# Autodesk Inventor assembly: Geeetech GT9S2 Extruder
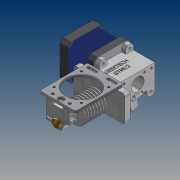
[picture p0: Inventor's stored thumbnail of the model, 180x180]
Saved by Autodesk Inventor 2019 (Build 230136000, 136)
## iProperties
Created: 2018-11-15
Part Number: Geeetech GT9S2 Extruder
Document SubType Name: Assembly
Designer: LillaHunden
Author: LillaHunden
## Documents named in this file (17)
- C:\Users\LillaHunden\Documents\Inventor\3dprinter\3dPrinter\Geeetech GT9S2 Extruder\Geeetech GT9S2 Extruder.iam
- C:\Users\LillaHunden\Documents\Inventor\3dprinter\3dPrinter\Geeetech GT9S2 Extruder\Cooling fin.ipt
- C:\Users\LillaHunden\Documents\Inventor\3dprinter\3dPrinter\Geeetech GT9S2 Extruder\extruder body.ipt
- C:\Users\LillaHunden\Documents\Inventor\3dprinter\3dPrinter\Geeetech GT9S2 Extruder\fan bracket.ipt
- C:\Users\LillaHunden\Documents\Inventor\3dprinter\3dPrinter\Geeetech GT9S2 Extruder\feeder tube.ipt
- C:\Users\LillaHunden\Documents\Inventor\3dprinter\3dPrinter\Geeetech GT9S2 Extruder\hotend.ipt
- C:\Users\LillaHunden\Documents\Inventor\3dprinter\3dPrinter\Geeetech GT9S2 Extruder\nozzel.ipt
- C:\Users\LillaHunden\Documents\Inventor\3dprinter\3dPrinter\Geeetech GT9S2 Extruder\Geeetech GT9S2 Extruder\Design Accelerator\Bolted Connection1.iam
- C:\Users\LillaHunden\Documents\Inventor\3dprinter\3dPrinter\Geeetech GT9S2 Extruder\Geeetech GT9S2 Extruder\Design Accelerator\Bolted Connection2.iam
- C:\Users\LillaHunden\Documents\Inventor\3dprinter\3dPrinter\Geeetech GT9S2 Extruder\roller bracket.ipt
- C:\Users\LillaHunden\Documents\Inventor\3dprinter\3dPrinter\Geeetech GT9S2 Extruder\roller bearing.ipt
- C:\Users\LillaHunden\Documents\Inventor\3dprinter\3dPrinter\Geeetech GT9S2 Extruder\roller pin.ipt
- C:\Users\LillaHunden\Documents\Inventor\3dprinter\3dPrinter\Geeetech GT9S2 Extruder\roller.ipt
- C:\Users\LillaHunden\Documents\Inventor\3dprinter\3dPrinter\Nema17 import\Nema 17HS4401-S.ipt
- C:\Users\LillaHunden\Documents\Inventor\3dprinter\3dPrinter\Geeetech GT9S2 Extruder\Geeetech GT9S2 Extruder\Design Accelerator\Bolted Connection3.iam
- C:\Users\LillaHunden\Documents\Inventor\3dprinter\3dPrinter\Geeetech GT9S2 Extruder\Fillament hob.ipt
- C:\Users\LillaHunden\Documents\Inventor\3dprinter\3dPrinter\Geeetech GT9S2 Extruder\fillament guide screw.ipt
## Components (16 placed, 14 different names)
1. Cooling fin:1 — Mate:5, Mate:6
2. extruder body:1 — Mate:1, Mate:2, Mate:9, Mate:17, Angle:3, Mate:18, Mate:19, Insert:1, Mate:22, Mate:23
3. fan bracket:1 — Mate:9, Angle:1, Angle:2, Flush:1, Mate:10, Mate:12
4. feeder tube:1 — Mate:1, Mate:2, Mate:3, Mate:4, Mate:5, Mate:6
5. hotend:1 — Mate:7, Mate:8, Angle:1, Angle:2, Flush:1, Mate:11, Mate:13
6. nozzel:1 — Mate:3, Mate:4, Mate:7, Mate:8
7. Bolted Connection:1 [sub-assembly] — Mate:10, Mate:11
8. Bolted Connection:2 [sub-assembly] — Mate:12, Mate:13
9. roller bracket:1 — Mate:16, Insert:1
10. roller bearing:1 — Mate:14, Flush:2, Mate:15
11. roller pin:1 — Mate:15, Mate:16
12. roller:1 — Mate:14, Flush:2
13. Nema 17HS4401-S:1 — Mate:17, Angle:3, Mate:18, Mate:20, Angle:4, Angle:5, Tangent:1, Mate:21
14. Bolted Connection:3 [sub-assembly] — Mate:19, Mate:20
15. Fillament hob:1 — Angle:4, Angle:5, Tangent:1, Mate:21
16. fillament guide screw:1 — Mate:22, Mate:23
## Relationships (32: Mate 23, Angle 5, Flush 2, Insert 1, Tangent 1)
- Mate:1: extruder body:1 ↔ feeder tube:1
- Mate:2 (1.35 mm): extruder body:1 ↔ feeder tube:1
- Mate:3: feeder tube:1 ↔ nozzel:1
- Mate:4 (0.3 mm): feeder tube:1 ↔ nozzel:1
- Mate:5: Cooling fin:1 ↔ feeder tube:1
- Mate:6 (4 mm): Cooling fin:1 ↔ feeder tube:1
- Mate:7: hotend:1 ↔ nozzel:1
- Mate:8: hotend:1 ↔ nozzel:1
- Mate:9: extruder body:1 ↔ fan bracket:1
- Angle:1 (0 deg): fan bracket:1 ↔ hotend:1
- Angle:2 (180 deg): fan bracket:1 ↔ hotend:1
- Flush:1: fan bracket:1 ↔ hotend:1
- Mate:10: fan bracket:1 ↔ Bolted Connection:1
- Mate:11: hotend:1 ↔ Bolted Connection:1
- Mate:12: fan bracket:1 ↔ Bolted Connection:2
- Mate:13: hotend:1 ↔ Bolted Connection:2
- Mate:14: roller bearing:1 ↔ roller:1
- Flush:2 (-0.5 mm): roller bearing:1 ↔ roller:1
- Mate:15: roller bearing:1 ↔ roller pin:1
- Mate:16: roller bracket:1 ↔ roller pin:1
- Mate:17: extruder body:1 ↔ Nema 17HS4401-S:1
- Angle:3 (0 deg): extruder body:1 ↔ Nema 17HS4401-S:1
- Mate:18: extruder body:1 ↔ Nema 17HS4401-S:1
- Mate:19: extruder body:1 ↔ Bolted Connection:3
- Mate:20: Nema 17HS4401-S:1 ↔ Bolted Connection:3
- Insert:1: extruder body:1 ↔ roller bracket:1
- Angle:4 (180 deg): Nema 17HS4401-S:1 ↔ Fillament hob:1
- Angle:5 (180 deg): Nema 17HS4401-S:1 ↔ Fillament hob:1
- Tangent:1: Nema 17HS4401-S:1 ↔ Fillament hob:1
- Mate:21 (6 mm): Nema 17HS4401-S:1 ↔ Fillament hob:1
- Mate:22: extruder body:1 ↔ fillament guide screw:1
- Mate:23: extruder body:1 ↔ fillament guide screw:1
